# Autodesk Inventor assembly: FRC100-1S
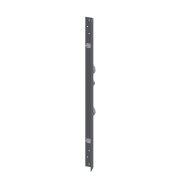
[picture p0: Inventor's stored thumbnail of the model, 180x180]
Saved by Autodesk Inventor 2020 (Build 240168000, 168)
## iProperties
Created: 2020-02-20
Part Number: FRC100-1S
Document SubType Name: Weldment
Designer: Juan Carlos Botero
Weld Material: Welded Aluminum-6061
Mass: 371.871 g
Surface Area: 2691.46 cm^2
Volume: 350.575 cm^3
Density: 1.06075 g/cm^3
Author: Juan Carlos Botero
Title: BARRA DE FRENO
## Documents named in this file (7)
- D:\Drives\OneDrive\Carlos_2\02 TRABAJOS\MULTIPLO\Conveyor\ENSAMBLE - Copy\Barra freno_W.iam
- D:\Drives\OneDrive\Carlos_2\02 TRABAJOS\MULTIPLO\Conveyor\ENSAMBLE\L Profile.ipt
- D:\Drives\OneDrive\Carlos_2\02 TRABAJOS\MULTIPLO\Conveyor\ENSAMBLE\Hook support_2.ipt
- D:\Drives\OneDrive\Carlos_2\02 TRABAJOS\MULTIPLO\Conveyor\ENSAMBLE\Eje de accionamiento freno.ipt
- D:\Drives\OneDrive\Carlos_2\02 TRABAJOS\MULTIPLO\Conveyor\ENSAMBLE\Solid1.ipt
- D:\Drives\OneDrive\Carlos_2\02 TRABAJOS\MULTIPLO\Conveyor\ENSAMBLE - Copy\Zapata_freno.ipt
- D:\Drives\OneDrive\Carlos_2\02 TRABAJOS\MULTIPLO\Conveyor\ENSAMBLE - Copy\Zapata_freno_MIR.ipt
## Components (10 placed, 6 different names)
1. L Profile:1 — Mate:1, Mate:2, Mate:3, Mate:4, Flush:1, Flush:2, Mate:5, Mate:6, Mate:7, Mate:8, Mate:9, Mate:10, Flush:3, Flush:4, Flush:5, Mate:11, Mate:12, Flush:6, Mate:13, Flush:7
2. Hook support_2:1 — Mate:1, Mate:3, Flush:1
3. Hook support_2:2 — Mate:2, Mate:4, Flush:2
4. Eje de accionamiento freno:1 — Mate:5, Mate:6, Flush:3
5. Solid1:1 — Mate:7, Mate:8, Flush:4
6. Solid1:2 — Mate:9, Mate:10, Flush:5
7. Zapata_freno:1 — Mate:11, Mate:12, Flush:6, Mate:14
8. Zapata_freno:2 — Mate:13, Flush:7, Mate:14
9. Zapata_freno_MIR:1 — Mate:15
10. Zapata_freno_MIR:2 — Mate:15
## Relationships (22: Mate 15, Flush 7)
- Mate:1: L Profile:1 ↔ Hook support_2:1
- Mate:2: L Profile:1 ↔ Hook support_2:2
- Mate:3: L Profile:1 ↔ Hook support_2:1
- Mate:4: L Profile:1 ↔ Hook support_2:2
- Flush:1 (200 mm): L Profile:1 ↔ Hook support_2:1
- Flush:2 (-200 mm): L Profile:1 ↔ Hook support_2:2
- Mate:5: L Profile:1 ↔ Eje de accionamiento freno:1
- Mate:6: L Profile:1 ↔ Eje de accionamiento freno:1
- Mate:7: L Profile:1 ↔ Solid1:1
- Mate:8: L Profile:1 ↔ Solid1:1
- Mate:9: L Profile:1 ↔ Solid1:2
- Mate:10: L Profile:1 ↔ Solid1:2
- Flush:3 (490 mm): L Profile:1 ↔ Eje de accionamiento freno:1
- Flush:4 (-400 mm): L Profile:1 ↔ Solid1:1
- Flush:5 (400 mm): L Profile:1 ↔ Solid1:2
- Mate:11: L Profile:1 ↔ Zapata_freno:1
- Mate:12 (6.35 mm): L Profile:1 ↔ Zapata_freno:1
- Flush:6: L Profile:1 ↔ Zapata_freno:1
- Mate:13: L Profile:1 ↔ Zapata_freno:2
- Flush:7: L Profile:1 ↔ Zapata_freno:2
- Mate:14: Zapata_freno:1 ↔ Zapata_freno:2
- Mate:15: Zapata_freno_MIR:1 ↔ Zapata_freno_MIR:2
